# Autodesk Inventor assembly: encoder_m_MIR1
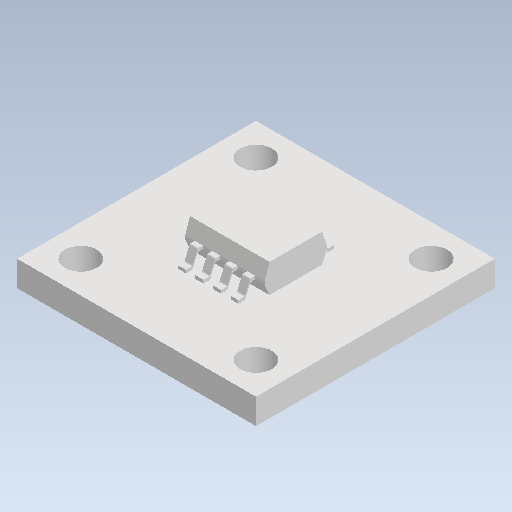
[picture p0: Inventor's stored thumbnail of the model, 512x512]
Saved by Autodesk Inventor 2020 (Build 240168000, 168)
## iProperties
Created: 2019-05-15
Part Number: encoder_m_MIR1
Document SubType Name: Assembly
Designer: psrob
Author: psrob
## Documents named in this file (3)
- E:\projects-2\project dog gen2\hardware\encoder_m_MIR1.iam
- E:\projects-2\project dog gen2\hardware\encoder_pcb_MIR.ipt
- E:\projects-2\project dog gen2\hardware\as5600_MIR.ipt
## Components (2 placed, 2 different names)
1. encoder_pcb_MIR:1 — Flush:2, Flush:1, Mate:1
2. as5600_MIR:1 — Flush:2, Flush:1, Mate:1
## Relationships (3: Flush 2, Mate 1)
- Flush:2 (4.5 mm): encoder_pcb_MIR:1 ↔ as5600_MIR:1
- Flush:1 (5 mm): encoder_pcb_MIR:1 ↔ as5600_MIR:1
- Mate:1: encoder_pcb_MIR:1 ↔ as5600_MIR:1
